# Autodesk Inventor assembly: Storage Assembly
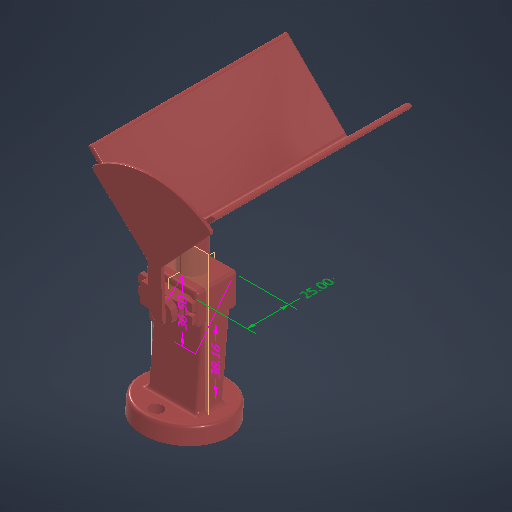
[picture p0: Inventor's stored thumbnail of the model, 512x512]
Saved by Autodesk Inventor 2026.2 (Build 302298010, 298A)
## iProperties
Created: 2026-04-14
Part Number: Storage Assembly
Document SubType Name: Assembly
Designer: lenovo
Author: lenovo
## Documents named in this file (4)
- C:\Users\lenovo\Downloads\storage 2\storage\Storage Assembly.iam
- C:\Users\lenovo\Downloads\storage 2\storage\Part1#2 .ipt
- C:\Users\lenovo\Downloads\storage 2\storage\Servo housing.ipt
- C:\Users\lenovo\Downloads\storage 2\storage\Part1_sG90.ipt
## Components (3 placed, 3 different names)
1. Part1#2 :1 — Mate:4, Mate:5
2. Servo housing:1 — Mate:1, Mate:2, Mate:3, Mate:5
3. Part1_sG90:1 — Mate:1, Mate:2, Mate:3, Mate:4
## Relationships (5: Mate 5)
- Mate:1: Servo housing:1 ↔ Part1_sG90:1
- Mate:2: Servo housing:1 ↔ Part1_sG90:1
- Mate:3: Servo housing:1 ↔ Part1_sG90:1
- Mate:4: Part1#2 :1 ↔ Part1_sG90:1
- Mate:5: Part1#2 :1 ↔ Servo housing:1
## Named parameters: Finish1_Area = 505.756, Finish1_Thickness = 0.05 mm
note: some values were not read from the file. Shown as the stored number, unit unknown: "Finish1_Area".
